# Autodesk Inventor assembly: Assembly
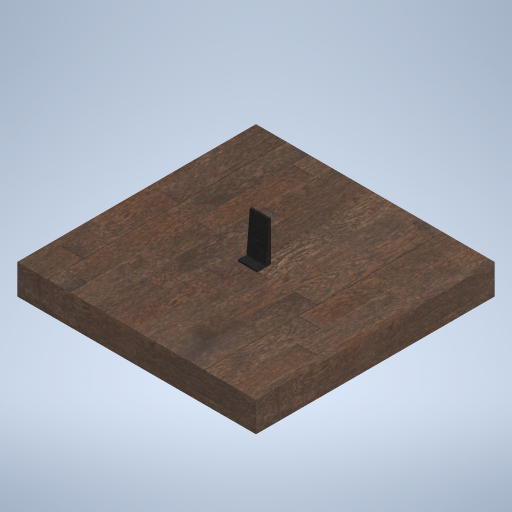
[picture p0: Inventor's stored thumbnail of the model, 512x512]
Saved by Autodesk Inventor 2023 (Build 270158000, 158)
## iProperties
Created: 2023-02-16
Part Number: Assembly
Document SubType Name: Assembly
Designer: shrey
Author: shrey
## Documents named in this file (3)
- D:\Inventor Projects\book stands\manga display\Assembly.iam
- D:\Inventor Projects\book stands\manga display\tabletop.ipt
- D:\Inventor Projects\book stands\manga display\stand.ipt
## Components (2 placed, 2 different names)
1. tabletop:1 — Mate:1, Mate:2, Flush:1
2. stand:1 — Mate:3, Mate:4, Flush:2
## Relationships (6: Mate 4, Flush 2)
- Mate:1: tabletop:1
- Mate:2: tabletop:1
- Flush:1: tabletop:1
- Mate:3: stand:1
- Mate:4: stand:1
- Flush:2: stand:1
